# Autodesk Inventor assembly: spur_gear_m0.8-18.4
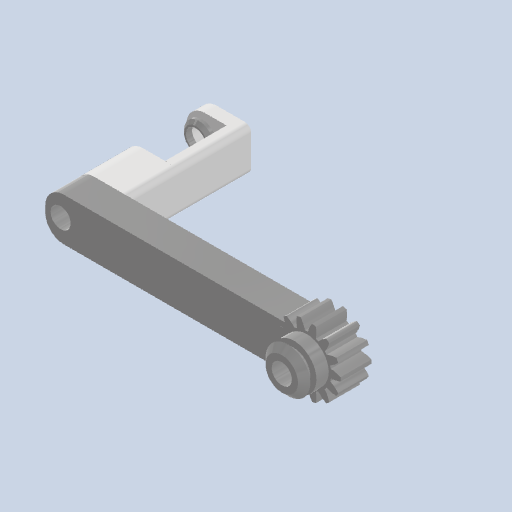
[picture p0: Inventor's stored thumbnail of the model, 512x512]
Saved by Autodesk Inventor 2025 (Build 290162000, 162)
## iProperties
Created: 2025-09-11
Part Number: spur_gear_m0.8-18.4
Document SubType Name: Assembly
Designer: sooo1
Author: sooo1
## Documents named in this file (7)
- C:\Users\sooo1\Documents\Inventor\MOBITOUCH\final\stroke_module_1\link_arm2_2.iam
- C:\Users\sooo1\Documents\Inventor\MOBITOUCH\final\stroke_module_1\平歯車1.iam
- C:\Users\sooo1\Documents\Inventor\MOBITOUCH\final\stroke_module_1\link_arm1_2.iam
- C:\Users\sooo1\Documents\Inventor\MOBITOUCH\final\stroke_module_1\spacer_Φ3.27_1.ipt
- C:\Users\sooo1\Documents\Inventor\MOBITOUCH\final\stroke_module_1\spacer_link.ipt
- C:\Users\sooo1\Documents\Inventor\MOBITOUCH\final\stroke_module_1\guide_link_2.ipt
- C:\Users\sooo1\Documents\Inventor\MOBITOUCH\final\stroke_module_1\spacer_Φ3.2_5.ipt
## Components (7 placed, 6 different names)
1. 平歯車:1 [sub-assembly] — 角度:7, フラッシュ:9, メイト:4
2. link_arm1_2:1 [sub-assembly] — メイト:1, フラッシュ:8, メイト:3, フラッシュ:9, メイト:4, メイト:5, メイト:6, フラッシュ:10, メイト:13, メイト:14
3. spacer_link:1 — メイト:5, メイト:6, フラッシュ:10, メイト:7, メイト:8, フラッシュ:11, メイト:11, メイト:12
4. guide_link_2:1 — メイト:7, メイト:8, フラッシュ:11, メイト:9, メイト:10
5. spacer_Φ3.27_1:1 — メイト:11, メイト:12
6. spacer_Φ3.27_1:2 — メイト:9, メイト:10
7. spacer_Φ3.2_5:1 — メイト:13, メイト:14
## Relationships (18: Mate 13, Flush 4, Angle 1)
- 角度:7 [Angle] (90 deg): 平歯車:1
- メイト:1 [Mate]: link_arm1_2:1
- フラッシュ:8 [Flush]: link_arm1_2:1
- メイト:3 [Mate]: link_arm1_2:1
- フラッシュ:9 [Flush]: 平歯車:1 ↔ link_arm1_2:1
- メイト:4 [Mate]: 平歯車:1 ↔ link_arm1_2:1
- メイト:5 [Mate]: link_arm1_2:1 ↔ spacer_link:1
- メイト:6 [Mate]: link_arm1_2:1 ↔ spacer_link:1
- フラッシュ:10 [Flush]: link_arm1_2:1 ↔ spacer_link:1
- メイト:7 [Mate]: spacer_link:1 ↔ guide_link_2:1
- メイト:8 [Mate]: spacer_link:1 ↔ guide_link_2:1
- フラッシュ:11 [Flush]: spacer_link:1 ↔ guide_link_2:1
- メイト:9 [Mate]: guide_link_2:1 ↔ spacer_Φ3.27_1:2
- メイト:10 [Mate]: guide_link_2:1 ↔ spacer_Φ3.27_1:2
- メイト:11 [Mate]: spacer_link:1 ↔ spacer_Φ3.27_1:1
- メイト:12 [Mate]: spacer_link:1 ↔ spacer_Φ3.27_1:1
- メイト:13 [Mate]: link_arm1_2:1 ↔ spacer_Φ3.2_5:1
- メイト:14 [Mate]: link_arm1_2:1 ↔ spacer_Φ3.2_5:1
